# Autodesk Inventor assembly: Camera_mount_v05
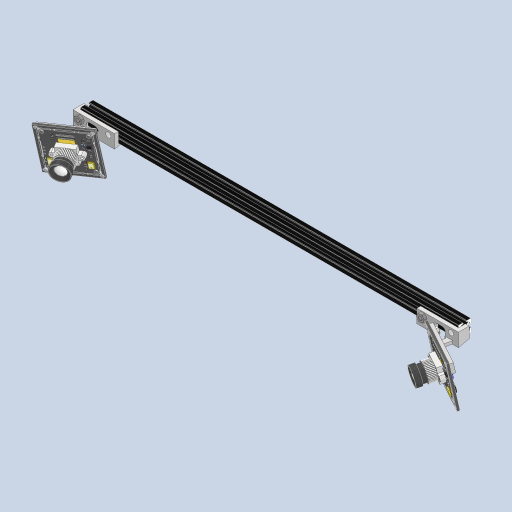
[picture p0: Inventor's stored thumbnail of the model, 512x512]
Saved by Autodesk Inventor 2024.4 (Build 284460000, 460)
## iProperties
Created: 2026-04-06
Part Number: Camera_mount_v05
Document SubType Name: Assembly
Designer: tooles01
Author: tooles01
## Documents named in this file (5)
- C:\Users\tooles01\NYU Langone Health Dropbox\Shannon Toole\Shannon_Dropbox\Mar lab\RFID\CAD\Camera_mount_angled\Camera_mount_v05.iam
- C:\Users\tooles01\NYU Langone Health Dropbox\Shannon Toole\Shannon_Dropbox\Mar lab\Inventor_Lib\100078 MB BE BL 300mm.ipt
- C:\Users\tooles01\NYU Langone Health Dropbox\Shannon Toole\Shannon_Dropbox\Mar lab\RFID\CAD\Camera_mount_angled\mount_05.iam
- C:\Users\tooles01\Documents\Inventor\Content Center Files\R2024\en-US\AS 1112 (2)\AS 1112 - M2  Type 5.ipt
- C:\Users\tooles01\NYU Langone Health Dropbox\Shannon Toole\Shannon_Dropbox\Mar lab\RFID\CAD\Camera_mount_angled\mount_05_mirror.iam
## Components (4 placed, 4 different names)
1. 100078 MB BE BL 300mm:1 — angle piece flush to post:1, angle piece to post end:1, angle piece to post bottom:1, angle piece flush to post:2, angle piece flush to post end:2, angle piece to post bottom:2
2. mount_05:1 [sub-assembly] — camera nut to angle piece, angle piece flush to post:1, angle piece to post end:1, angle piece to post bottom:1
3. mount_05_mirror:1 [sub-assembly] — angle piece flush to post:2, angle piece flush to post end:2, angle piece to post bottom:2
4. AS 1112 (2) - Metric M2  Type 5:1 — camera nut to angle piece
## Relationships (7: Mate 6, Insert 1)
- camera nut to angle piece [Insert]: mount_05:1 ↔ AS 1112 (2) - Metric M2  Type 5:1
- angle piece flush to post:1 [Mate]: 100078 MB BE BL 300mm:1 ↔ mount_05:1
- angle piece to post end:1 [Mate]: 100078 MB BE BL 300mm:1 ↔ mount_05:1
- angle piece to post bottom:1 [Mate]: 100078 MB BE BL 300mm:1 ↔ mount_05:1
- angle piece flush to post:2 [Mate]: 100078 MB BE BL 300mm:1 ↔ mount_05_mirror:1
- angle piece flush to post end:2 [Mate]: 100078 MB BE BL 300mm:1 ↔ mount_05_mirror:1
- angle piece to post bottom:2 [Mate]: 100078 MB BE BL 300mm:1 ↔ mount_05_mirror:1
